# Autodesk Inventor assembly: Typewriter
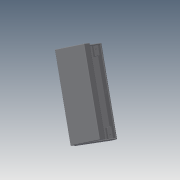
[picture p0: Inventor's stored thumbnail of the model, 180x180]
Saved by Autodesk Inventor 2019 (Build 230136000, 136)
## iProperties
Created: 2019-07-03
Part Number: Typewriter
Document SubType Name: Assembly
Designer: giacomo
Author: giacomo
## Documents named in this file (4)
- D:\Hobby\Inventor\Case 3Dprinted\Typewriter.iam
- D:\Hobby\Inventor\Case 3Dprinted\A\CaseA.iam
- D:\Hobby\Inventor\Case 3Dprinted\B\Case B.iam
- D:\Hobby\Inventor\Prove 3D printer\Cerniera\Definitiva\Cerniera_definitiva.iam
## Components (4 placed, 3 different names)
1. CaseA:1 [sub-assembly] — Mate:1, Mate:2, Mate:3, Mate:4, Mate:9, Mate:11
2. Case B:1 [sub-assembly] — Mate:8, Mate:12, Mate:13, Mate:14, Mate:15, Mate:16
3. Cerniera_definitiva:1 [sub-assembly] — Mate:1, Mate:2, Mate:11, Mate:12, Mate:13, Mate:14
4. Cerniera_definitiva:2 [sub-assembly] — Mate:3, Mate:4, Mate:8, Mate:9, Mate:15, Mate:16
## Relationships (12: Mate 12)
- Mate:1: CaseA:1 ↔ Cerniera_definitiva:1
- Mate:2: CaseA:1 ↔ Cerniera_definitiva:1
- Mate:3: CaseA:1 ↔ Cerniera_definitiva:2
- Mate:4: CaseA:1 ↔ Cerniera_definitiva:2
- Mate:8: Case B:1 ↔ Cerniera_definitiva:2
- Mate:9: CaseA:1 ↔ Cerniera_definitiva:2
- Mate:11: CaseA:1 ↔ Cerniera_definitiva:1
- Mate:12: Case B:1 ↔ Cerniera_definitiva:1
- Mate:13: Case B:1 ↔ Cerniera_definitiva:1
- Mate:14: Case B:1 ↔ Cerniera_definitiva:1
- Mate:15: Case B:1 ↔ Cerniera_definitiva:2
- Mate:16: Case B:1 ↔ Cerniera_definitiva:2
